# Autodesk Inventor assembly: 6v dc torque motor_MIR
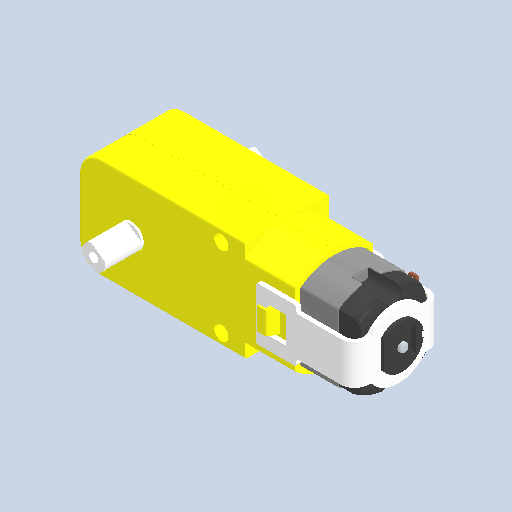
[picture p0: Inventor's stored thumbnail of the model, 512x512]
Saved by Autodesk Inventor 2023.2 (Build 272271000, 271)
## iProperties
Company: Unknown
Created: 2022-10-12
Part Number: 6v dc torque motor_MIR
Description: Unknown
Document SubType Name: Assembly
Designer: omrfrkmll
Title: Moteur
Author: Unknown
Sending System: DEX
Preprocessor: ST-DEVELOPER v16.7
## Documents named in this file (11)
- C:\Users\omr_f\Desktop\mechanism design project\6v dc torque motor_MIR.iam
- C:\Users\omr_f\Desktop\mechanism design project\Moteur - Enveloppe partie 1 _MIR.ipt
- C:\Users\omr_f\Desktop\mechanism design project\Moteur - Engrenage 1_MIR.ipt
- C:\Users\omr_f\Desktop\mechanism design project\Moteur - Engrenage 2_MIR.ipt
- C:\Users\omr_f\Desktop\mechanism design project\Moteur - Moteur_MIR.ipt
- C:\Users\omr_f\Desktop\mechanism design project\Moteur - Axe engrenage_MIR.ipt
- C:\Users\omr_f\Desktop\mechanism design project\Moteur - Vis_MIR.ipt
- C:\Users\omr_f\Desktop\mechanism design project\Moteur - Enveloppe partie 2_MIR.ipt
- C:\Users\omr_f\Desktop\mechanism design project\Moteur - Maintien_MIR.ipt
- C:\Users\omr_f\Desktop\mechanism design project\Moteur - Engrenage 3_MIR.ipt
- C:\Users\omr_f\Desktop\mechanism design project\Moteur - Engrenage 4_MIR.ipt
## Components (11 placed, 10 different names)
1. Moteur - Enveloppe partie 1 _MIR:1 — Mate:2, Mate:1
2. Moteur - Engrenage 1_MIR:1 — Mate:2, Mate:1
3. Moteur - Engrenage 2_MIR:1
4. Moteur - Moteur_MIR:1
5. Moteur - Axe engrenage_MIR:1
6. Moteur - Vis_MIR:1
7. Moteur - Vis_MIR:2
8. Moteur - Enveloppe partie 2_MIR:1
9. Moteur - Maintien_MIR:1
10. Moteur - Engrenage 3_MIR:1
11. Moteur - Engrenage 4_MIR:1
## Relationships (2: Mate 2)
- Mate:2: Moteur - Enveloppe partie 1 _MIR:1 ↔ Moteur - Engrenage 1_MIR:1
- Mate:1: Moteur - Enveloppe partie 1 _MIR:1 ↔ Moteur - Engrenage 1_MIR:1
